# Autodesk Inventor assembly: Assembly1
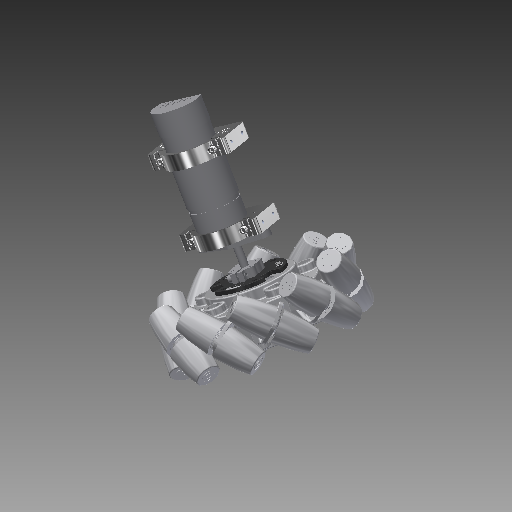
[picture p0: Inventor's stored thumbnail of the model, 512x512]
Saved by Autodesk Inventor 2017 (Build 210142000, 142)
## iProperties
Created: 2017-09-20
Part Number: Assembly1
Document SubType Name: Assembly
Designer: User
Author: User
## Documents named in this file (7)
- C:\Robotics\CAD\2017-18_CAD\DirectDriveMotorSubAsembly.iam
- C:\Robotics\CAD\COTSParts\Vex\6inchMecanumRight217-2586-STEP\6inchMecanumRight217-2586.20121203.ipt
- C:\Robotics\CAD\COTSParts\Vex\VersaHub.5inchBore217-4009-STEP-20140807\VersaHub.5inchBore217-4009-STEP-20140807.ipt
- C:\Robotics\CAD\COTSParts\Motors\Andymark 2964  NeveRest 40 Motor.ipt
- C:\Robotics\CAD\COTSParts\Actobotics\545 parts\545618 clamping hub.ipt
- C:\Robotics\CAD\COTSParts\Tetrix\tetrix-motor-mounts-1.snapshot.1\Tetrex 2pc motor mount.ipt
- C:\Robotics\CAD\2017-18_CAD\MotorFixedPositionMount17_18.ipt
## Components (7 placed, 6 different names)
1. 6inchMecanumRight217-2586.20121203:3
2. VersaHub.5inchBore217-4009-STEP-20140807:2 — Mate:24
3. Andymark 2964  NeveRest 40 Motor:2 — Mate:25, Flush:5, Mate:26, Mate:27, Mate:29
4. 545618 clamping hub:2 — Mate:24
5. Tetrex 2pc motor mount:1 — Mate:26, Flush:28, Flush:29
6. Tetrex 2pc motor mount:2 — Mate:25, Flush:5, Flush:28, Flush:29, Mate:28
7. MotorFixedPositionMount17_18:1 — Mate:27, Mate:28, Mate:29
## Relationships (15: Mate 11, Flush 4)
- [Mate]: 6inchMecanumRight217-2586.20121203:3 ↔ VersaHub.5inchBore217-4009-STEP-20140807:2
- [Mate]: 6inchMecanumRight217-2586.20121203:3 ↔ VersaHub.5inchBore217-4009-STEP-20140807:2
- [Mate]: 6inchMecanumRight217-2586.20121203:3 ↔ VersaHub.5inchBore217-4009-STEP-20140807:2
- [Mate]: Andymark 2964  NeveRest 40 Motor:2 ↔ 545618 clamping hub:2
- [Flush]: Andymark 2964  NeveRest 40 Motor:2 ↔ 545618 clamping hub:2
- [Mate]: VersaHub.5inchBore217-4009-STEP-20140807:2 ↔ Andymark 2964  NeveRest 40 Motor:2
- Mate:24: VersaHub.5inchBore217-4009-STEP-20140807:2 ↔ 545618 clamping hub:2
- Mate:25: Andymark 2964  NeveRest 40 Motor:2 ↔ Tetrex 2pc motor mount:2
- Flush:5: Andymark 2964  NeveRest 40 Motor:2 ↔ Tetrex 2pc motor mount:2
- Mate:26: Andymark 2964  NeveRest 40 Motor:2 ↔ Tetrex 2pc motor mount:1
- Flush:28 (60.0456 mm): Tetrex 2pc motor mount:1 ↔ Tetrex 2pc motor mount:2
- Flush:29: Tetrex 2pc motor mount:1 ↔ Tetrex 2pc motor mount:2
- Mate:27: Andymark 2964  NeveRest 40 Motor:2 ↔ MotorFixedPositionMount17_18:1
- Mate:28: Tetrex 2pc motor mount:2 ↔ MotorFixedPositionMount17_18:1
- Mate:29: Andymark 2964  NeveRest 40 Motor:2 ↔ MotorFixedPositionMount17_18:1
## Named parameters: d30_d25 = 0 mm, d31_d26 = 0 mm, d33_d29 = 0 mm, d34_d11 = 0 mm, d35_d12 = 0 mm, d37_d15 = 0 mm
